# Autodesk Inventor assembly: spur_gear_m0.8-18.4
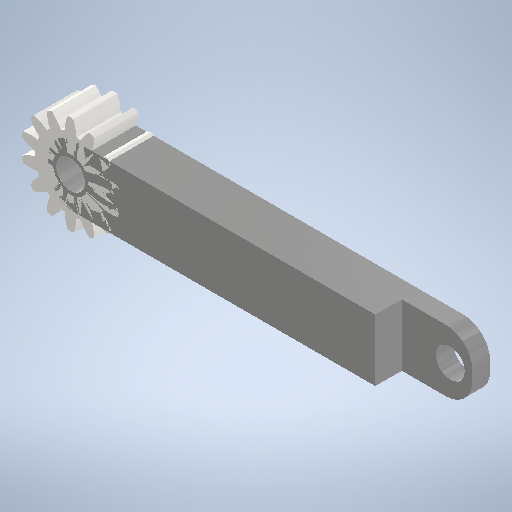
[picture p0: Inventor's stored thumbnail of the model, 512x512]
Saved by Autodesk Inventor 2025 (Build 290162000, 162)
## iProperties
Created: 2025-09-11
Part Number: spur_gear_m0.8-18.4
Document SubType Name: Assembly
Designer: sooo1
Author: sooo1
## Documents named in this file (3)
- C:\Users\sooo1\Documents\Inventor\MOBITOUCH\final\stroke_module_1\link_arm_p2.iam
- C:\Users\sooo1\Documents\Inventor\MOBITOUCH\final\stroke_module_1\link_arm_b2.ipt
- C:\Users\sooo1\Documents\Inventor\MOBITOUCH\final\stroke_module_1\平歯車1.iam
## Components (2 placed, 2 different names)
1. link_arm_b2:1 — フラッシュ:1, フラッシュ:2, フラッシュ:3, フラッシュ:4, 角度:1
2. 平歯車:1 [sub-assembly] — フラッシュ:4, 角度:1
## Relationships (5: Flush 4, Angle 1)
- フラッシュ:1 [Flush]: link_arm_b2:1
- フラッシュ:2 [Flush]: link_arm_b2:1
- フラッシュ:3 [Flush]: link_arm_b2:1
- フラッシュ:4 [Flush]: link_arm_b2:1 ↔ 平歯車:1
- 角度:1 [Angle] (0 deg): link_arm_b2:1 ↔ 平歯車:1
